# Autodesk Inventor assembly: Instrumentboardhousing
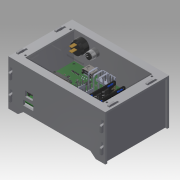
[picture p0: Inventor's stored thumbnail of the model, 180x180]
Saved by Autodesk Inventor 2019.3 (Build 233278000, 278)
## iProperties
Created: 2019-05-28
Part Number: Instrumentboardhousing
Document SubType Name: Assembly
Designer: Dave
Author: Dave
## Documents named in this file (13)
- C:\Users\Dave\Dropbox\ProjectODMeter\HousingCAD\Instrumentboardhousing.iam
- C:\Users\Dave\Dropbox\ProjectODMeter\HousingCAD\bottom_instrumentboard.ipt
- C:\Users\Dave\Dropbox\ProjectODMeter\HousingCAD\motorcontroller.ipt
- C:\Users\Dave\Dropbox\ProjectODMeter\HousingCAD\top_instrumentboard.ipt
- C:\Users\Dave\Dropbox\ProjectODMeter\HousingCAD\TouchScreen.ipt
- C:\Users\Dave\Dropbox\ProjectODMeter\HousingCAD\ODMeter.ipt
- C:\Users\Dave\Dropbox\ProjectODMeter\HousingCAD\front_instrumentboard.ipt
- C:\Users\Dave\Dropbox\ProjectODMeter\HousingCAD\back_instrumentboard.ipt
- C:\Users\Dave\Dropbox\ProjectODMeter\HousingCAD\sides_instreamentboard.ipt
- C:\Users\Dave\Dropbox\ProjectODMeter\HousingCAD\6pin.ipt
- C:\Users\Dave\Dropbox\ProjectODMeter\HousingCAD\barrel_plug.ipt
- C:\Users\Dave\Dropbox\ProjectODMeter\HousingCAD\pwr_btn.ipt
- C:\Users\Dave\Dropbox\ProjectODMeter\HousingCAD\standoff.ipt
## Components (20 placed, 12 different names)
1. bottom_instrumentboard:1 — Mate:4, Mate:5, Mate:6, Mate:7, Mate:8, Mate:9, Mate:10, Mate:11, Mate:12, Mate:33, Mate:34, Mate:35, Mate:36, Mate:37, Mate:38, Mate:39, Mate:40, Mate:41, Mate:42, Mate:43, Mate:44
2. top_instrumentboard:1 — Mate:1, Mate:2, Mate:3, Mate:13, Mate:14, Mate:15, Mate:16, Mate:17, Mate:18, Mate:19, Mate:20
3. TouchScreen:1 — Mate:1, Mate:2, Mate:3
4. ODMeter:1 — Mate:4, Mate:5, Mate:6
5. front_instrumentboard:1 — Mate:7, Mate:8, Mate:9, Mate:16, Mate:25, Mate:26, Mate:27, Mate:28, Mate:29, Mate:30, Mate:31, Mate:32
6. back_instrumentboard:1 — Mate:10, Mate:11, Mate:12, Mate:13, Mate:14, Mate:15
7. sides_instreamentboard:1 — Mate:18, Mate:19
8. sides_instreamentboard:2 — Mate:17, Mate:20
9. motorcontroller:1 — Mate:21, Mate:23, Flush:1, Mate:46, Mate:49, Mate:51
10. motorcontroller:2 — Mate:21, Mate:22, Mate:23, Mate:24, Flush:1, Flush:2, Mate:50, Mate:52
11. motorcontroller:3 — Mate:22, Mate:24, Flush:2, Mate:45, Mate:47, Mate:48
12. 6pin:1 — Mate:25, Mate:26, Mate:27
13. barrel_plug:1 — Mate:31, Mate:32
14. pwr_btn:1 — Mate:28, Mate:29, Mate:30
15. standoff:1 — Mate:33, Mate:39, Mate:46, Mate:51
16. standoff:2 — Mate:34, Mate:42, Mate:49
17. standoff:3 — Mate:35, Mate:40, Mate:52
18. standoff:4 — Mate:36, Mate:43, Mate:50
19. standoff:5 — Mate:37, Mate:41, Mate:45, Mate:47
20. standoff:6 — Mate:38, Mate:44, Mate:48
## Relationships (54: Mate 52, Flush 2)
- Mate:1: top_instrumentboard:1 ↔ TouchScreen:1
- Mate:2: top_instrumentboard:1 ↔ TouchScreen:1
- Mate:3: top_instrumentboard:1 ↔ TouchScreen:1
- Mate:4: bottom_instrumentboard:1 ↔ ODMeter:1
- Mate:5: bottom_instrumentboard:1 ↔ ODMeter:1
- Mate:6 (5 mm): bottom_instrumentboard:1 ↔ ODMeter:1
- Mate:7: bottom_instrumentboard:1 ↔ front_instrumentboard:1
- Mate:8: bottom_instrumentboard:1 ↔ front_instrumentboard:1
- Mate:9: bottom_instrumentboard:1 ↔ front_instrumentboard:1
- Mate:10: bottom_instrumentboard:1 ↔ back_instrumentboard:1
- Mate:11: bottom_instrumentboard:1 ↔ back_instrumentboard:1
- Mate:12: bottom_instrumentboard:1 ↔ back_instrumentboard:1
- Mate:13: top_instrumentboard:1 ↔ back_instrumentboard:1
- Mate:14: top_instrumentboard:1 ↔ back_instrumentboard:1
- Mate:15: top_instrumentboard:1 ↔ back_instrumentboard:1
- Mate:16: top_instrumentboard:1 ↔ front_instrumentboard:1
- Mate:17: top_instrumentboard:1 ↔ sides_instreamentboard:2
- Mate:18: top_instrumentboard:1 ↔ sides_instreamentboard:1
- Mate:19: top_instrumentboard:1 ↔ sides_instreamentboard:1
- Mate:20: top_instrumentboard:1 ↔ sides_instreamentboard:2
- Mate:21: motorcontroller:1 ↔ motorcontroller:2
- Mate:22: motorcontroller:2 ↔ motorcontroller:3
- Mate:23: motorcontroller:1 ↔ motorcontroller:2
- Mate:24: motorcontroller:2 ↔ motorcontroller:3
- Flush:1 (15 mm): motorcontroller:1 ↔ motorcontroller:2
- Flush:2 (15 mm): motorcontroller:2 ↔ motorcontroller:3
- Mate:25: front_instrumentboard:1 ↔ 6pin:1
- Mate:26: front_instrumentboard:1 ↔ 6pin:1
- Mate:27: front_instrumentboard:1 ↔ 6pin:1
- Mate:28: front_instrumentboard:1 ↔ pwr_btn:1
- Mate:29: front_instrumentboard:1 ↔ pwr_btn:1
- Mate:30: front_instrumentboard:1 ↔ pwr_btn:1
- Mate:31: front_instrumentboard:1 ↔ barrel_plug:1
- Mate:32: front_instrumentboard:1 ↔ barrel_plug:1
- Mate:33: bottom_instrumentboard:1 ↔ standoff:1
- Mate:34: bottom_instrumentboard:1 ↔ standoff:2
- Mate:35: bottom_instrumentboard:1 ↔ standoff:3
- Mate:36: bottom_instrumentboard:1 ↔ standoff:4
- Mate:37: bottom_instrumentboard:1 ↔ standoff:5
- Mate:38: bottom_instrumentboard:1 ↔ standoff:6
- Mate:39: bottom_instrumentboard:1 ↔ standoff:1
- Mate:40: bottom_instrumentboard:1 ↔ standoff:3
- Mate:41: bottom_instrumentboard:1 ↔ standoff:5
- Mate:42: bottom_instrumentboard:1 ↔ standoff:2
- Mate:43: bottom_instrumentboard:1 ↔ standoff:4
- Mate:44: bottom_instrumentboard:1 ↔ standoff:6
- Mate:45: motorcontroller:3 ↔ standoff:5
- Mate:46: motorcontroller:1 ↔ standoff:1
- Mate:47: motorcontroller:3 ↔ standoff:5
- Mate:48: motorcontroller:3 ↔ standoff:6
- Mate:49: motorcontroller:1 ↔ standoff:2
- Mate:50: motorcontroller:2 ↔ standoff:4
- Mate:51: motorcontroller:1 ↔ standoff:1
- Mate:52: motorcontroller:2 ↔ standoff:3
